# Autodesk Inventor assembly: Kevin_CAD_test_assembly
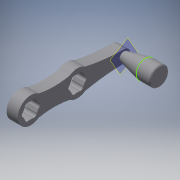
[picture p0: Inventor's stored thumbnail of the model, 180x180]
Saved by Autodesk Inventor 2016 (Build 200138000, 138)
## iProperties
Created: 2018-06-19
Part Number: Kevin_CAD_test_assembly
Document SubType Name: Assembly
Designer: Student
Author: Student
## Documents named in this file (3)
- C:\Users\Student\Documents\Derek Code and Projects\Autodesk\Kevin_CAD_test_assembly.iam
- C:\Users\Student\Documents\Derek Code and Projects\Autodesk\Kevin_CAD_test.ipt
- C:\Users\Student\Documents\Derek Code and Projects\Autodesk\Kevin_CAD_test_2.ipt
## Components (2 placed, 2 different names)
1. Kevin_CAD_test:1 — Rotational:1
2. Kevin_CAD_test_2:1 — Rotational:1
## Relationships (1: RevoluteJoint 1)
- Rotational:1 [RevoluteJoint]: Kevin_CAD_test:1 ↔ Kevin_CAD_test_2:1
